# Autodesk Inventor assembly: XCarriageFanTop.old
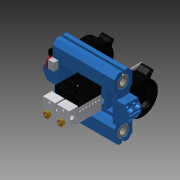
[picture p0: Inventor's stored thumbnail of the model, 180x180]
Saved by Autodesk Inventor 2015 SP1 (Build 190203100, 203)
## iProperties
Created: 2014-12-10
Part Number: XCarriageFanTop.old
Document SubType Name: Assembly
Designer: Jack
Author: Jack
## Documents named in this file (8)
- C:\Users\Jack\ownCloud\Projects\CoreXY\InventorModel\XAxis\XCarriageFanTop.old.iam
- C:\Users\Jack\ownCloud\Projects\CoreXY\InventorModel\HotEnds\E3DChimera\E3DChimera.iam
- C:\Users\Jack\ownCloud\Projects\CoreXY\InventorModel\Electronics\Fans\FanRadial40mm.ipt
- C:\Users\Jack\ownCloud\Projects\CoreXY\InventorModel\XAxis\ChimeraXCarriage3.ipt
- C:\Users\Jack\ownCloud\Projects\CoreXY\InventorModel\XAxis\XCarriageFanMount.ipt
- C:\Users\Jack\ownCloud\Projects\CoreXY\InventorModel\Electronics\EndStops\EndStopOptical.ipt
- C:\Users\Jack\ownCloud\Projects\CoreXY\InventorModel\Hardware\Bearing\BearingLinear\BearingLinearLMU8.ipt
- C:\Users\Jack\ownCloud\Projects\CoreXY\InventorModel\XAxis\XCarriageBeltClipRound.ipt
## Components (14 placed, 7 different names)
1. E3DChimera:1 [sub-assembly]
2. FanRadial40mm:1
3. FanRadial40mm:2
4. ChimeraXCarriage3:1 — Mate:27, Flush:2, Mate:28, Mate:29, Mate:30, Flush:3, Flush:4, Flush:5, Mate:31, Mate:32, Mate:33, Mate:34, Mate:35, Mate:36, Mate:37, Mate:38, Mate:39, Mate:40, Mate:41, Mate:42
5. XCarriageFanMount:1
6. EndStopOptical:1
7. BearingLinearLMU8:1 — Mate:27, Flush:2
8. BearingLinearLMU8:2 — Mate:28, Flush:5
9. BearingLinearLMU8:3 — Mate:30, Flush:3
10. BearingLinearLMU8:4 — Mate:29, Flush:4
11. XCarriageBeltClipRound:1 — Mate:31, Mate:32, Mate:33
12. XCarriageBeltClipRound:2 — Mate:34, Mate:35, Mate:36
13. XCarriageBeltClipRound:3 — Mate:37, Mate:39, Mate:40
14. XCarriageBeltClipRound:4 — Mate:38, Mate:41, Mate:42
## Relationships (37: Mate 29, Flush 5, Angle 3)
- [Angle] (180 deg): E3DChimera:1 ↔ FanRadial40mm:2
- [Angle] (180 deg): E3DChimera:1 ↔ FanRadial40mm:1
- [Flush]: FanRadial40mm:1 ↔ FanRadial40mm:2
- [Mate]: E3DChimera:1 ↔ ChimeraXCarriage3:1
- [Mate]: E3DChimera:1 ↔ ChimeraXCarriage3:1
- [Mate]: FanRadial40mm:2 ↔ ChimeraXCarriage3:1
- [Mate]: FanRadial40mm:2 ↔ ChimeraXCarriage3:1
- [Mate]: FanRadial40mm:1 ↔ ChimeraXCarriage3:1
- [Mate]: FanRadial40mm:1 ↔ ChimeraXCarriage3:1
- [Mate]: FanRadial40mm:2 ↔ ChimeraXCarriage3:1
- [Mate]: E3DChimera:1 ↔ ChimeraXCarriage3:1
- [Mate]: ChimeraXCarriage3:1 ↔ XCarriageFanMount:1
- [Mate]: ChimeraXCarriage3:1 ↔ XCarriageFanMount:1
- [Mate]: FanRadial40mm:2 ↔ XCarriageFanMount:1
- [Mate]: ChimeraXCarriage3:1 ↔ EndStopOptical:1
- [Angle] (180 deg): ChimeraXCarriage3:1 ↔ EndStopOptical:1
- [Mate]: ChimeraXCarriage3:1 ↔ EndStopOptical:1
- Mate:27: ChimeraXCarriage3:1 ↔ BearingLinearLMU8:1
- Flush:2: ChimeraXCarriage3:1 ↔ BearingLinearLMU8:1
- Mate:28: ChimeraXCarriage3:1 ↔ BearingLinearLMU8:2
- Mate:29: ChimeraXCarriage3:1 ↔ BearingLinearLMU8:4
- Mate:30: ChimeraXCarriage3:1 ↔ BearingLinearLMU8:3
- Flush:3: ChimeraXCarriage3:1 ↔ BearingLinearLMU8:3
- Flush:4: ChimeraXCarriage3:1 ↔ BearingLinearLMU8:4
- Flush:5: ChimeraXCarriage3:1 ↔ BearingLinearLMU8:2
- Mate:31: ChimeraXCarriage3:1 ↔ XCarriageBeltClipRound:1
- Mate:32: ChimeraXCarriage3:1 ↔ XCarriageBeltClipRound:1
- Mate:33: ChimeraXCarriage3:1 ↔ XCarriageBeltClipRound:1
- Mate:34: ChimeraXCarriage3:1 ↔ XCarriageBeltClipRound:2
- Mate:35: ChimeraXCarriage3:1 ↔ XCarriageBeltClipRound:2
- Mate:36: ChimeraXCarriage3:1 ↔ XCarriageBeltClipRound:2
- Mate:37: ChimeraXCarriage3:1 ↔ XCarriageBeltClipRound:3
- Mate:38: ChimeraXCarriage3:1 ↔ XCarriageBeltClipRound:4
- Mate:39: ChimeraXCarriage3:1 ↔ XCarriageBeltClipRound:3
- Mate:40: ChimeraXCarriage3:1 ↔ XCarriageBeltClipRound:3
- Mate:41: ChimeraXCarriage3:1 ↔ XCarriageBeltClipRound:4
- Mate:42: ChimeraXCarriage3:1 ↔ XCarriageBeltClipRound:4
